# Autodesk Inventor assembly: 1stCutAtChainDrivenSystem
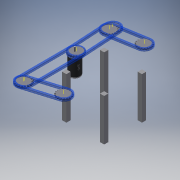
[picture p0: Inventor's stored thumbnail of the model, 180x180]
Saved by Autodesk Inventor 2016 SP1 (Build 200210100, 210)
## iProperties
Created: 2016-01-21
Part Number: 1stCutAtChainDrivenSystem
Document SubType Name: Assembly
Designer: steele
Author: steele
## Documents named in this file (7)
- C:\snobotics\CAD-Development\robSteele\SnoBotics2016\2ndCutAtPitchingMachineRobot\1stCutAtChainDrivenSystem.iam
- C:\snobotics\CAD-Development\robSteele\SnoBotics2016\2ndCutAtPitchingMachineRobot\VeryBasicFrame.ipt
- C:\snobotics\autodesk\2015\FRC_KOP_2015\Motors\MOT_CIM-Motor_217-2000.iam
- C:\snobotics\CAD-Development\robSteele\SnoBotics2016\2ndCutAtPitchingMachineRobot\1stCutAtChainDrivenSystem\Design Accelerator\Chain Drive1.iam
- C:\snobotics\CAD-Development\robSteele\SnoBotics2016\2ndCutAtPitchingMachineRobot\1stCutAtChainDrivenSystem\Design Accelerator\Chain Drive3.iam
- C:\snobotics\CAD-Development\robSteele\SnoBotics2016\2ndCutAtPitchingMachineRobot\1stCutAtChainDrivenSystem\Design Accelerator\Chain Drive4.iam
- C:\snobotics\CAD-Development\robSteele\SnoBotics2016\2ndCutAtPitchingMachineRobot\1stCutAtChainDrivenSystem\Design Accelerator\Chain Drive5.iam
## Components (6 placed, 3 different names)
1. VeryBasicFrame:1 — Flush:1, Flush:2
2. MOT_CIM-Motor_217-2000:1 [sub-assembly] — Flush:1, Mate:1, Flush:2
3. Chain Drive:1 [sub-assembly]
4. Chain Drive:2 [sub-assembly]
5. Chain Drive:3 [sub-assembly]
6. Chain Drive:4 [sub-assembly]
## Relationships (3: Flush 2, Mate 1)
- Flush:1: VeryBasicFrame:1 ↔ MOT_CIM-Motor_217-2000:1
- Mate:1: MOT_CIM-Motor_217-2000:1
- Flush:2: VeryBasicFrame:1 ↔ MOT_CIM-Motor_217-2000:1
